# Autodesk Inventor assembly: Crank_Slider_Fixer
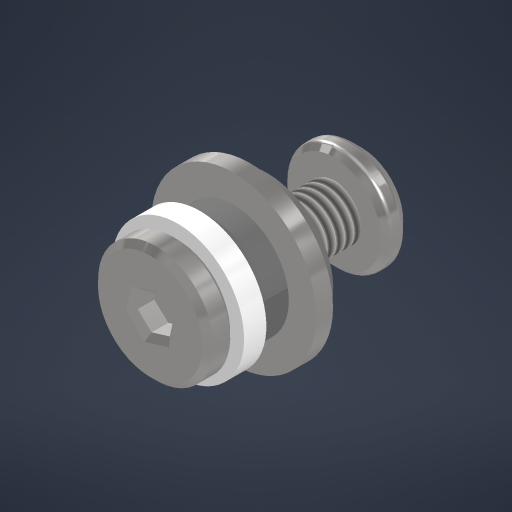
[picture p0: Inventor's stored thumbnail of the model, 512x512]
Saved by Autodesk Inventor 2024.3 (Build 283343000, 343)
## iProperties
Created: 2024-01-28
Part Number: Crank_Slider_Fixer
Document SubType Name: Assembly
Designer: 김대겸
Author: 김대겸
## Documents named in this file (5)
- C:\Users\ASUS\Desktop\Anti_Backlash_Structure_OP\MISUMI\Crank_Slider_Fixer.iam
- C:\Users\ASUS\Desktop\Anti_Backlash_Structure_OP\MISUMI\LED-0606.ipt
- C:\Users\ASUS\Desktop\Anti_Backlash_Structure_OP\v3_Frame\Ubber_Washer_1.5mm.ipt
- C:\Users\ASUS\Desktop\Anti_Backlash_Structure_OP\MISUMI\TT-0610-20.ipt
- C:\Users\ASUS\Desktop\Anti_Backlash_Structure_OP\V2_Frame(2025)\MISUMI\M5-D6-8mm.ipt
## Components (4 placed, 4 different names)
1. LED-0606:1 — 삽입:2, 삽입:4, 삽입:5
2. Ubber_Washer_1.5mm:4 — 삽입:2
3. TT-0610-20:1 — 삽입:4
4. M5-D6-8mm:1 — 삽입:5
## Relationships (3: Insert 3)
- 삽입:2 [Insert]: LED-0606:1 ↔ Ubber_Washer_1.5mm:4
- 삽입:4 [Insert]: LED-0606:1 ↔ TT-0610-20:1
- 삽입:5 [Insert]: LED-0606:1 ↔ M5-D6-8mm:1
